# Autodesk Inventor assembly: Assembly1
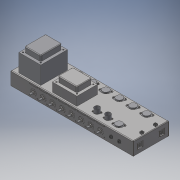
[picture p0: Inventor's stored thumbnail of the model, 180x180]
Saved by Autodesk Inventor 2016 (Build 200138000, 138)
## iProperties
Created: 2015-10-14
Part Number: Assembly1
Document SubType Name: Assembly
Designer: jeremyhale
Author: jeremyhale
## Documents named in this file (31)
- \\psf\Home\Documents\Poorhouse\git\p0001\chassis.iam
- chassis.iam
- \\psf\Home\Documents\Poorhouse\git\p0001\tube socket 8 pin.ipt
- \\psf\Home\Documents\Poorhouse\git\p0001\tube socket 9 pin.ipt
- \\psf\Home\Documents\Poorhouse\git\p0001\xmfr power.ipt
- \\psf\Home\Documents\Poorhouse\git\p0001\xmfr output.ipt
- \\psf\Home\Documents\Inventor\Content Center Files\R2016\en-US\AS 1427(08)\AS 1427 - M3 x 5(6) I.ipt
- \\psf\Home\Documents\Inventor\Content Center Files\R2016\en-US\AS 1474(1)\AS 1474 - M2.5(1).ipt
- \\psf\Home\Documents\Inventor\Content Center Files\R2016\en-US\AS 1474(1)\AS 1474 - M3.5(1).ipt
- \\psf\Home\Documents\Inventor\Content Center Files\R2016\en-US\AS 1474(1)\AS 1474 - M3(1).ipt
- \\psf\Home\Documents\Poorhouse\git\p0001\iec320_703W-00_04.ipt
- \\psf\Home\Documents\Inventor\Content Center Files\R2016\en-US\AS 1427(07)\AS 1427 - M3 x 10(6) II.ipt
- \\psf\Home\Documents\Poorhouse\git\p0001\Toggle Large A.ipt
- \\psf\Home\Documents\Poorhouse\git\p0001\AUDIO JACK 2.ipt
- \\psf\Home\Documents\Poorhouse\git\p0001\12ax7_complete.ipt
- \\psf\Home\Documents\Poorhouse\git\p0001\Noval socket.ipt
- \\psf\Home\Documents\Poorhouse\git\p0001\octal assembly.ipt
- \\psf\Home\Documents\Poorhouse\git\p0001\el34 assembly_r1.ipt
- \\psf\Home\Documents\Poorhouse\git\p0001\Bussman fuse holder HKP - 0,25'' X 1,25''.ipt
- \\psf\Home\Documents\Poorhouse\git\p0001\cage nut m6.iam
- \\psf\Home\Documents\Poorhouse\git\p0001\PEC11R-4220F-S0024.ipt
- \\psf\Home\Documents\Inventor\Content Center Files\R2016\en-US\UNI 5590  A\UNI 5590 - A M7.ipt
- \\psf\Home\Documents\Inventor\Content Center Files\R2016\en-US\BS 4320(2)\BS 4320 - M7 (Form B).ipt
- \\psf\Home\Documents\Poorhouse\git\p0001\rotary control.iam
- \\psf\Home\Documents\Poorhouse\git\p0001\Standoff 7mm M2 Wurth 9774070243R.ipt
- \\psf\Home\Documents\Poorhouse\git\p0001\chassis\Design Accelerator\Bolted Connection2.iam
- \\psf\Home\Documents\Poorhouse\git\p0001\chassis\Design Accelerator\Bolted Connection3.iam
- \\psf\Home\Documents\Poorhouse\git\p0001\chassis\Design Accelerator\Bolted Connection4.iam
- \\psf\Home\Documents\Poorhouse\git\p0001\chassis\Design Accelerator\Bolted Connection5.iam
- \\psf\Home\Documents\Poorhouse\git\p0001\chassis\Design Accelerator\Bolted Connection8.iam
- \\psf\Home\Documents\Poorhouse\git\p0001\chassis-weld.iam
## Components (216 placed, 28 different names)
1. big preamp tube sockets — Insert:13, Insert:14
2. xmfr power:1
3. xmfr output:1
4. Bussman fuse holder HKP - 0,25'' X 1,25'':1
5. PowerSwitch
6. chassis-weld:1 [sub-assembly] — Angle:1, Rotational:29
7. AS 1474 - Metric M2.5:1 — Mate:3
8. AS 1474 - Metric M3.5:1
9. AS 1474 - Metric M3.5:2
10. AS 1474 - Metric M3.5:3
11. AS 1474 - Metric M3.5:4
12. AS 1474 - Metric M3.5:5
13. AS 1474 - Metric M3.5:6
14. AS 1474 - Metric M3.5:7
15. AS 1474 - Metric M3.5:8
16. AS 1474 - Metric M3.5:9
17. AS 1474 - Metric M3.5:10
18. AS 1474 - Metric M3.5:11
19. AS 1474 - Metric M3.5:12
20. AS 1474 - Metric M3.5:13
21. AS 1474 - Metric M3.5:14
22. AS 1474 - Metric M3:1
23. AS 1474 - Metric M3:2
24. AS 1474 - Metric M3:3
25. AS 1474 - Metric M3:4
26. AS 1427 Z - Metric M3 x 5:1 — Insert:1, Mate:3
27. AS 1427 Z - Metric M3 x 5:2 — Insert:2
28. AS 1427 Z - Metric M3 x 5:3 — Insert:3
29. AS 1427 Z - Metric M3 x 5:4 — Insert:4
30. AS 1427 Z - Metric M3 x 5:5 — Insert:5
31. AS 1427 Z - Metric M3 x 5:6 — Insert:6
32. AS 1427 Z - Metric M3 x 5:7 — Insert:7
33. AS 1427 Z - Metric M3 x 5:8 — Insert:8
34. AS 1427 Z - Metric M3 x 5:9 — Insert:9
35. AS 1427 Z - Metric M3 x 5:10 — Insert:10
36. AS 1427 Z - Metric M3 x 5:11 — Insert:11
37. AS 1427 Z - Metric M3 x 5:12 — Insert:12
38. AS 1427 Z - Metric M3 x 5:13 — Insert:13
39. AS 1427 Z - Metric M3 x 5:14 — Insert:14
40. AS 1427 Z - Metric M3 x 5:15 — Insert:15
41. AS 1427 Z - Metric M3 x 5:16 — Insert:16
42. AS 1427 Z - Metric M3 x 5:17 — Insert:17
43. AS 1427 Z - Metric M3 x 5:18 — Insert:18
44. iec320_703W-00_04:1 — Mate:6, Mate:7
45. AS 1427 Z - Metric M3 x 10:2 — Mate:6, Mate:10
46. AS 1427 Z - Metric M3 x 10:1 — Mate:7, Mate:12
47. AS 1474 - Metric M3:5 — Mate:10
48. AS 1474 - Metric M3:6 — Mate:12
49. 12ax7_complete:1 — Rotational:13
50. 12ax7_complete:2 — Rotational:14
51. Noval socket:1 — Rotational:13
52. Noval socket:2 — Rotational:14
53. octal assembly:1
54. octal assembly:2 — Rotational:21
55. octal assembly:3 — Rotational:22
56. octal assembly:4 — Rotational:23
57. octal assembly:5 — Rigid:21
58. octal assembly:6 — Rotational:24
59. octal assembly:7 — Rotational:25
60. el34 assembly_r1:1 — Rotational:21
61. el34 assembly_r1:2 — Rotational:22
62. el34 assembly_r1:3 — Rigid:21
63. el34 assembly_r1:4 — Rotational:23
64. el34 assembly_r1:5 — Rotational:24
65. el34 assembly_r1:6 — Rotational:25
66. tube socket 8 pin:1 — Insert:1, Insert:2
67. tube socket 8 pin:2 — Insert:3, Insert:4
68. tube socket 8 pin:3 — Insert:5, Insert:6
69. tube socket 8 pin:4 — Insert:7, Insert:8
70. tube socket 8 pin:5 — Insert:15, Insert:16
71. tube socket 8 pin:6 — Insert:17, Insert:18
72. tube socket 9 pin:1 — Insert:9, Insert:10
73. tube socket 9 pin:2 — Insert:11, Insert:12
74. Speaker
75. AUDIO JACK 2:3
76. AUDIO JACK 2:4
77. cage nut m6:1 [sub-assembly]
78. cage nut m6:2 [sub-assembly]
79. cage nut m6:3 [sub-assembly]
80. cage nut m6:4 [sub-assembly]
81. cage nut m6:5 [sub-assembly]
82. cage nut m6:6 [sub-assembly]
83. cage nut m6:7 [sub-assembly]
84. cage nut m6:8 [sub-assembly]
85. Input Jack
86. AUDIO JACK 2:5
87. Bolted Connection:4 [sub-assembly] — Mate:38
88. Bolted Connection:3 [sub-assembly] — Mate:30
89. Bolted Connection:2 [sub-assembly] — Mate:32
90. Bolted Connection:1 [sub-assembly] — Mate:34
91. Standoff 7mm M2 Wurth 9774070243R:4 — Insert:42, Mate:38
92. Standoff 7mm M2 Wurth 9774070243R:3 — Insert:41, Mate:32
93. Standoff 7mm M2 Wurth 9774070243R:2 — Insert:40, Mate:30
94. Standoff 7mm M2 Wurth 9774070243R:1 — Insert:39, Mate:34
95. rotary control:1 [sub-assembly] — Insert:39, Insert:40, Insert:41, Insert:42, Angle:1, Cylindrical:1, Mate:39, Mate:40
96. BS 4320 Form AB M7 (Form B):1 — Mate:15, Mate:18
97. UNI 5590 A A M7:1 — Mate:17, Mate:18
98. PEC11R-4220F-S0024:1 — Mate:15, Mate:17, Cylindrical:1
99. Bolted Connection:37 [sub-assembly]
100. Bolted Connection:38 [sub-assembly]
101. Bolted Connection:39 [sub-assembly]
102. Bolted Connection:40 [sub-assembly]
103. Standoff 7mm M2 Wurth 9774070243R:5
104. Standoff 7mm M2 Wurth 9774070243R:6
105. Standoff 7mm M2 Wurth 9774070243R:7
106. Standoff 7mm M2 Wurth 9774070243R:8
107. rotary control:2 [sub-assembly]
108. BS 4320 Form AB M7 (Form B):2
109. UNI 5590 A A M7:2
110. PEC11R-4220F-S0024:2
111. Bolted Connection:45 [sub-assembly]
112. Bolted Connection:46 [sub-assembly]
113. Bolted Connection:47 [sub-assembly]
114. Bolted Connection:48 [sub-assembly]
115. Standoff 7mm M2 Wurth 9774070243R:9
116. Standoff 7mm M2 Wurth 9774070243R:10
117. Standoff 7mm M2 Wurth 9774070243R:11
118. Standoff 7mm M2 Wurth 9774070243R:12
119. rotary control:3 [sub-assembly]
120. BS 4320 Form AB M7 (Form B):3
121. UNI 5590 A A M7:3
122. PEC11R-4220F-S0024:3
123. Bolted Connection:53 [sub-assembly]
124. Bolted Connection:54 [sub-assembly]
125. Bolted Connection:55 [sub-assembly]
126. Bolted Connection:56 [sub-assembly]
127. Standoff 7mm M2 Wurth 9774070243R:13
128. Standoff 7mm M2 Wurth 9774070243R:14
129. Standoff 7mm M2 Wurth 9774070243R:15
130. Standoff 7mm M2 Wurth 9774070243R:16
131. rotary control:4 [sub-assembly]
132. BS 4320 Form AB M7 (Form B):4
133. UNI 5590 A A M7:4
134. PEC11R-4220F-S0024:4
135. Bolted Connection:61 [sub-assembly]
136. Bolted Connection:62 [sub-assembly]
137. Bolted Connection:63 [sub-assembly]
138. Bolted Connection:64 [sub-assembly]
139. Standoff 7mm M2 Wurth 9774070243R:17
140. Standoff 7mm M2 Wurth 9774070243R:18
141. Standoff 7mm M2 Wurth 9774070243R:19
142. Standoff 7mm M2 Wurth 9774070243R:20
143. rotary control:5 [sub-assembly]
144. BS 4320 Form AB M7 (Form B):5
145. UNI 5590 A A M7:5
146. PEC11R-4220F-S0024:5
147. Bolted Connection:69 [sub-assembly]
148. Bolted Connection:70 [sub-assembly]
149. Bolted Connection:71 [sub-assembly]
150. Bolted Connection:72 [sub-assembly]
151. Standoff 7mm M2 Wurth 9774070243R:21
152. Standoff 7mm M2 Wurth 9774070243R:22
153. Standoff 7mm M2 Wurth 9774070243R:23
154. Standoff 7mm M2 Wurth 9774070243R:24
155. rotary control:6 [sub-assembly]
156. BS 4320 Form AB M7 (Form B):6
157. UNI 5590 A A M7:6
158. PEC11R-4220F-S0024:6
159. Bolted Connection:77 [sub-assembly]
160. Bolted Connection:78 [sub-assembly]
161. Bolted Connection:79 [sub-assembly]
162. Bolted Connection:80 [sub-assembly]
163. Standoff 7mm M2 Wurth 9774070243R:25
164. Standoff 7mm M2 Wurth 9774070243R:26
165. Standoff 7mm M2 Wurth 9774070243R:27
166. Standoff 7mm M2 Wurth 9774070243R:28
167. rotary control:7 [sub-assembly]
168. BS 4320 Form AB M7 (Form B):7
169. UNI 5590 A A M7:7
170. PEC11R-4220F-S0024:7
171. Bolted Connection:85 [sub-assembly]
172. Bolted Connection:86 [sub-assembly]
173. Bolted Connection:87 [sub-assembly]
174. Bolted Connection:88 [sub-assembly]
175. Standoff 7mm M2 Wurth 9774070243R:29
176. Standoff 7mm M2 Wurth 9774070243R:30
177. Standoff 7mm M2 Wurth 9774070243R:31
178. Standoff 7mm M2 Wurth 9774070243R:32
179. rotary control:8 [sub-assembly]
180. BS 4320 Form AB M7 (Form B):8
181. UNI 5590 A A M7:8
182. PEC11R-4220F-S0024:8
183. AUDIO JACK 2:6 — Rotational:29
184. AUDIO JACK 2:7
185. Bolted Connection:33 [sub-assembly] — Mate:39, Mate:40
186. Bolted Connection:34 [sub-assembly]
187. Bolted Connection:35 [sub-assembly]
188. Bolted Connection:36 [sub-assembly]
189. Bolted Connection:41 [sub-assembly]
190. Bolted Connection:42 [sub-assembly]
191. Bolted Connection:43 [sub-assembly]
192. Bolted Connection:44 [sub-assembly]
193. Bolted Connection:49 [sub-assembly]
194. Bolted Connection:50 [sub-assembly]
195. Bolted Connection:51 [sub-assembly]
196. Bolted Connection:52 [sub-assembly]
197. Bolted Connection:57 [sub-assembly]
198. Bolted Connection:58 [sub-assembly]
199. Bolted Connection:59 [sub-assembly]
200. Bolted Connection:60 [sub-assembly]
201. Bolted Connection:65 [sub-assembly]
202. Bolted Connection:66 [sub-assembly]
203. Bolted Connection:67 [sub-assembly]
204. Bolted Connection:68 [sub-assembly]
205. Bolted Connection:73 [sub-assembly]
206. Bolted Connection:74 [sub-assembly]
207. Bolted Connection:75 [sub-assembly]
208. Bolted Connection:76 [sub-assembly]
209. Bolted Connection:81 [sub-assembly]
210. Bolted Connection:82 [sub-assembly]
211. Bolted Connection:83 [sub-assembly]
212. Bolted Connection:84 [sub-assembly]
213. Bolted Connection:89 [sub-assembly]
214. Bolted Connection:90 [sub-assembly]
215. Bolted Connection:91 [sub-assembly]
216. Bolted Connection:92 [sub-assembly]
## Component patterns: Big Tube Sockets (6 elements), small preamp tube sockets (2 elements), jacks speaker (3 elements), Cage Nuts Top (4 elements), Cage Nuts Right (2 elements), Cage Nuts Left (2 elements), jacks input (2 elements), controls (8 elements), jacks fx (2 elements), (4 elements, first: Bolted Connection:33), Component Pattern 21:2 (4 elements), Component Pattern 21:3 (4 elements), Component Pattern 21:4 (4 elements), Component Pattern 21:5 (4 elements), Component Pattern 21:6 (4 elements), Component Pattern 21:7 (4 elements), Component Pattern 21:8 (4 elements)
## Relationships (107: Insert 40, RevoluteJoint 28, Mate 24, WeldJoint 10, Flush 3, Angle 1, CylindricalJoint 1)
- [RevoluteJoint]: chassis-weld:1 ↔ tube socket 8 pin:1
- [RevoluteJoint]: chassis-weld:1 ↔ tube socket 8 pin:1
- [RevoluteJoint]: big preamp tube sockets ↔ chassis-weld:1
- [RevoluteJoint]: big preamp tube sockets ↔ chassis-weld:1
- [RevoluteJoint]: chassis-weld:1 ↔ tube socket 9 pin:1
- [RevoluteJoint]: chassis-weld:1 ↔ tube socket 9 pin:1
- [RevoluteJoint]: xmfr power:1 ↔ chassis-weld:1
- [RevoluteJoint]: xmfr power:1 ↔ chassis-weld:1
- [RevoluteJoint]: xmfr output:1 ↔ chassis-weld:1
- [RevoluteJoint]: xmfr output:1 ↔ chassis-weld:1
- Insert:1: AS 1427 Z - Metric M3 x 5:1 ↔ tube socket 8 pin:1
- Insert:2: AS 1427 Z - Metric M3 x 5:2 ↔ tube socket 8 pin:1
- Insert:3: AS 1427 Z - Metric M3 x 5:3 ↔ tube socket 8 pin:2
- Insert:4: AS 1427 Z - Metric M3 x 5:4 ↔ tube socket 8 pin:2
- Insert:5: AS 1427 Z - Metric M3 x 5:5 ↔ tube socket 8 pin:3
- Insert:6: AS 1427 Z - Metric M3 x 5:6 ↔ tube socket 8 pin:3
- Insert:7: AS 1427 Z - Metric M3 x 5:7 ↔ tube socket 8 pin:4
- Insert:8: AS 1427 Z - Metric M3 x 5:8 ↔ tube socket 8 pin:4
- Insert:9: AS 1427 Z - Metric M3 x 5:9 ↔ tube socket 9 pin:1
- Insert:10: AS 1427 Z - Metric M3 x 5:10 ↔ tube socket 9 pin:1
- Insert:11: AS 1427 Z - Metric M3 x 5:11 ↔ tube socket 9 pin:2
- Insert:12: AS 1427 Z - Metric M3 x 5:12 ↔ tube socket 9 pin:2
- Insert:13: big preamp tube sockets ↔ AS 1427 Z - Metric M3 x 5:13
- Insert:14: big preamp tube sockets ↔ AS 1427 Z - Metric M3 x 5:14
- Insert:15: AS 1427 Z - Metric M3 x 5:15 ↔ tube socket 8 pin:5
- Insert:16: AS 1427 Z - Metric M3 x 5:16 ↔ tube socket 8 pin:5
- Insert:17: AS 1427 Z - Metric M3 x 5:17 ↔ tube socket 8 pin:6
- Insert:18: AS 1427 Z - Metric M3 x 5:18 ↔ tube socket 8 pin:6
- Mate:3: AS 1474 - Metric M2.5:1 ↔ AS 1427 Z - Metric M3 x 5:1
- [Mate]: chassis-weld:1 ↔ AS 1474 - Metric M2.5:1
- [Insert]: chassis-weld:1 ↔ AS 1474 - Metric M3.5:1
- [Insert]: chassis-weld:1 ↔ AS 1474 - Metric M3.5:2
- [Insert]: chassis-weld:1 ↔ AS 1474 - Metric M3.5:3
- [Insert]: chassis-weld:1 ↔ AS 1474 - Metric M3.5:4
- [Insert]: chassis-weld:1 ↔ AS 1474 - Metric M3.5:5
- [Insert]: chassis-weld:1 ↔ AS 1474 - Metric M3.5:6
- [Insert]: chassis-weld:1 ↔ AS 1474 - Metric M3.5:7
- [Insert]: chassis-weld:1 ↔ AS 1474 - Metric M3.5:8
- [Insert]: chassis-weld:1 ↔ AS 1474 - Metric M3.5:9
- [Insert]: chassis-weld:1 ↔ AS 1474 - Metric M3.5:10
- [Insert]: chassis-weld:1 ↔ AS 1474 - Metric M3.5:11
- [Insert]: chassis-weld:1 ↔ AS 1474 - Metric M3.5:12
- [Insert]: chassis-weld:1 ↔ AS 1474 - Metric M3.5:13
- [Insert]: chassis-weld:1 ↔ AS 1474 - Metric M3.5:14
- [Insert]: chassis-weld:1 ↔ AS 1474 - Metric M3:1
- [Insert]: chassis-weld:1 ↔ AS 1474 - Metric M3:2
- [Insert]: chassis-weld:1 ↔ AS 1474 - Metric M3:3
- [Insert]: chassis-weld:1 ↔ AS 1474 - Metric M3:4
- [RevoluteJoint]: chassis-weld:1 ↔ iec320_703W-00_04:1
- [RevoluteJoint]: chassis-weld:1 ↔ iec320_703W-00_04:1
- Mate:6: iec320_703W-00_04:1 ↔ AS 1427 Z - Metric M3 x 10:2
- Mate:7: iec320_703W-00_04:1 ↔ AS 1427 Z - Metric M3 x 10:1
- Mate:10: AS 1427 Z - Metric M3 x 10:2 ↔ AS 1474 - Metric M3:5
- [Mate]: chassis-weld:1 ↔ AS 1474 - Metric M3:5
- Mate:12: AS 1427 Z - Metric M3 x 10:1 ↔ AS 1474 - Metric M3:6
- [Mate]: chassis-weld:1 ↔ AS 1474 - Metric M3:6
- [WeldJoint]: chassis-weld:1 ↔ Speaker
- [WeldJoint]: chassis-weld:1 ↔ Noval socket:1
- [WeldJoint]: chassis-weld:1 ↔ Noval socket:2
- Rotational:13 [RevoluteJoint]: 12ax7_complete:1 ↔ Noval socket:1
- Rotational:14 [RevoluteJoint]: 12ax7_complete:2 ↔ Noval socket:2
- [WeldJoint]: chassis-weld:1 ↔ octal assembly:1
- [RevoluteJoint]: chassis-weld:1 ↔ octal assembly:2
- [RevoluteJoint]: chassis-weld:1 ↔ octal assembly:3
- [RevoluteJoint]: chassis-weld:1 ↔ octal assembly:5
- [RevoluteJoint]: chassis-weld:1 ↔ octal assembly:4
- [RevoluteJoint]: chassis-weld:1 ↔ octal assembly:6
- [RevoluteJoint]: chassis-weld:1 ↔ octal assembly:7
- Rotational:21 [RevoluteJoint]: octal assembly:2 ↔ el34 assembly_r1:1
- Rotational:22 [RevoluteJoint]: octal assembly:3 ↔ el34 assembly_r1:2
- Rigid:21 [WeldJoint]: octal assembly:5 ↔ el34 assembly_r1:3
- Rotational:23 [RevoluteJoint]: octal assembly:4 ↔ el34 assembly_r1:4
- Rotational:24 [RevoluteJoint]: octal assembly:6 ↔ el34 assembly_r1:5
- Rotational:25 [RevoluteJoint]: octal assembly:7 ↔ el34 assembly_r1:6
- [WeldJoint]: Bussman fuse holder HKP - 0,25'' X 1,25'':1 ↔ chassis-weld:1
- [WeldJoint]: PowerSwitch ↔ chassis-weld:1
- [Flush]: chassis-weld:1
- [Flush]: chassis-weld:1
- [Flush]: chassis-weld:1
- [WeldJoint]: chassis-weld:1 ↔ cage nut m6:1
- [WeldJoint]: chassis-weld:1 ↔ cage nut m6:5
- [WeldJoint]: chassis-weld:1 ↔ cage nut m6:7
- Mate:15: BS 4320 Form AB M7 (Form B):1 ↔ PEC11R-4220F-S0024:1
- [Mate]: chassis-weld:1 ↔ BS 4320 Form AB M7 (Form B):1
- Mate:17: UNI 5590 A A M7:1 ↔ PEC11R-4220F-S0024:1
- Mate:18: BS 4320 Form AB M7 (Form B):1 ↔ UNI 5590 A A M7:1
- Insert:39: Standoff 7mm M2 Wurth 9774070243R:1 ↔ rotary control:1
- Insert:40: Standoff 7mm M2 Wurth 9774070243R:2 ↔ rotary control:1
- Insert:41: Standoff 7mm M2 Wurth 9774070243R:3 ↔ rotary control:1
- Insert:42: Standoff 7mm M2 Wurth 9774070243R:4 ↔ rotary control:1
- [Mate]: chassis-weld:1 ↔ Standoff 7mm M2 Wurth 9774070243R:1
- [Mate]: chassis-weld:1 ↔ Standoff 7mm M2 Wurth 9774070243R:4
- Angle:1 (0 deg): chassis-weld:1 ↔ rotary control:1
- Cylindrical:1: rotary control:1 ↔ PEC11R-4220F-S0024:1
- [Mate]: chassis-weld:1 ↔ Bolted Connection:3
- Mate:30: Bolted Connection:3 ↔ Standoff 7mm M2 Wurth 9774070243R:2
- [Mate]: chassis-weld:1 ↔ Bolted Connection:2
- Mate:32: Bolted Connection:2 ↔ Standoff 7mm M2 Wurth 9774070243R:3
- [Mate]: chassis-weld:1 ↔ Bolted Connection:1
- Mate:34: Bolted Connection:1 ↔ Standoff 7mm M2 Wurth 9774070243R:1
- [RevoluteJoint]: chassis-weld:1 ↔ Input Jack
- [RevoluteJoint]: chassis-weld:1 ↔ PEC11R-4220F-S0024:1
- [Mate]: chassis-weld:1 ↔ Bolted Connection:4
- Mate:38: Bolted Connection:4 ↔ Standoff 7mm M2 Wurth 9774070243R:4
- Mate:39: rotary control:1 ↔ Bolted Connection:33
- Mate:40: rotary control:1 ↔ Bolted Connection:33
- Rotational:29 [RevoluteJoint]: chassis-weld:1 ↔ AUDIO JACK 2:6
## Named parameters: ControlSpacing = 44.45 mm
